# Autodesk Inventor assembly: wheel
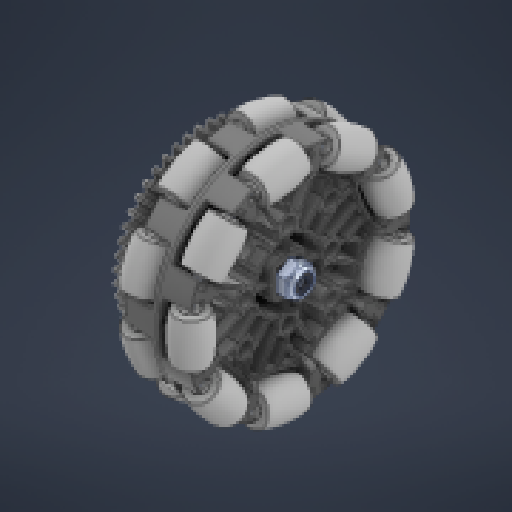
[picture p0: Inventor's stored thumbnail of the model, 512x512]
Saved by Autodesk Inventor 2024 (Build 280153000, 153)
## iProperties
Created: 2023-10-29
Part Number: wheel
Document SubType Name: Assembly
Designer: Averey Ku
Author: Averey Ku
## Documents named in this file (7)
- C:\Users\avere\Documents\rbp_cad\zoomba_v0.1\chassis\drivebay\wheel.iam
- C:\Users\avere\Documents\rbp_cad\VEX-CAD-Inventor-1.41\Motion\Wheels\Omni Wheel\2.75 Omni AS, No Insert.iam
- C:\Users\avere\Documents\rbp_cad\zoomba_v0.1\chassis\drivebay\custom_parts\ls_48t.ipt
- C:\Users\avere\Documents\rbp_cad\VEX-CAD-Inventor-1.41\Motion\Spacers\Spacer Nylon .500 OD\NSpacer White .500 OD x .250.ipt
- C:\Users\avere\Documents\rbp_cad\VEX-CAD-Inventor-1.41\Structure\Hardware\Nut Thin Nylock.ipt
- C:\Users\avere\Documents\rbp_cad\VEX-CAD-Inventor-1.41\Motion\Wheels\Omni Wheel.iam
- C:\Users\avere\Documents\rbp_cad\VEX-CAD-Inventor-1.41\Motion\Spacers\Spacer Nylon .500 OD.ipt
## Components (5 placed, 4 different names)
1. 2.75 Omni AS, No Insert:1 [sub-assembly] — Insert:9, Insert:14, Mate:1
2. ls_48t:1 — Insert:12, Insert:13
3. NSpacer White .500 OD x .250:1 — Insert:13, Insert:14
4. NSpacer White .500 OD x .250:2 — Insert:12, Mate:1
5. Nut Thin Nylock:1 — Insert:9
## Relationships (5: Insert 4, Mate 1)
- Insert:9: 2.75 Omni AS, No Insert:1 ↔ Nut Thin Nylock:1
- Insert:12: ls_48t:1 ↔ NSpacer White .500 OD x .250:2
- Insert:13: ls_48t:1 ↔ NSpacer White .500 OD x .250:1
- Insert:14: 2.75 Omni AS, No Insert:1 ↔ NSpacer White .500 OD x .250:1
- Mate:1: 2.75 Omni AS, No Insert:1 ↔ NSpacer White .500 OD x .250:2
